# Autodesk Inventor assembly: mecanum prototype
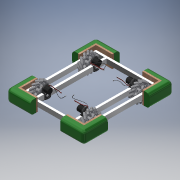
[picture p0: Inventor's stored thumbnail of the model, 180x180]
Saved by Autodesk Inventor 2018 (Build 220112000, 112)
## iProperties
Created: 2019-04-24
Part Number: mecanum prototype
Document SubType Name: Assembly
Designer: corbin
Sending System: Autodesk Inventor 2019
Preprocessor: ST-DEVELOPER v17
Title: C:\Users\corbin\Downloads\mecanum prototype.stp
Author: corbin
## Documents named in this file (10)
- C:\Users\corbin\Downloads\mecanum prototype\mecanum prototype.iam
- C:\Users\corbin\Downloads\mecanum prototype\parts\Frame Pieces\sides with bearings.iam
- C:\Users\corbin\Downloads\mecanum prototype\parts\Frame Pieces\front and back.ipt
- C:\Users\corbin\Downloads\mecanum prototype\parts\Gearbox\Single_Reduction_Clamping_Gearbox_217-4156.iam
- C:\Users\corbin\Downloads\mecanum prototype\parts\Churro.ipt
- C:\Users\corbin\Downloads\mecanum prototype\parts\REV-21-1650.ipt
- C:\Users\corbin\Downloads\mecanum prototype\parts\Wheels\8 Inch Mecanum Wheels\8_Mecanum_Wheel_Right_217-2587.iam
- C:\Users\corbin\Downloads\mecanum prototype\parts\Wheels\8 Inch Mecanum Wheels\8_Mecanum_Wheel_Left_217-2801.iam
- C:\Users\corbin\Downloads\mecanum prototype\parts\Frame Pieces\outsides.ipt
- C:\Users\corbin\Downloads\mecanum prototype\parts\bumpers.ipt
## Components (26 placed, 9 different names)
1. sides with bearings:1 [sub-assembly] — Flush:6, Mate:13, Mate:21, Mate:23, Mate:24, Mate:26, Mate:30, Flush:16, Mate:31, Flush:17
2. sides with bearings:4 [sub-assembly] — Mate:7, Flush:8, Mate:8, Flush:13, Mate:14, Mate:15, Mate:16, Mate:19, Mate:20, Mate:25, Mate:27, Mate:28, Flush:14, Mate:29, Flush:15
3. front and back:1 — Mate:6, Mate:7, Flush:8, Flush:9, Mate:11, Flush:12
4. front and back:2 — Mate:1, Flush:1, Flush:2, Mate:2, Flush:3, Flush:4, Mate:3, Flush:5, Flush:6, Flush:10, Mate:8, Mate:10, Flush:11, Flush:13
5. Single_Reduction_Clamping_Gearbox_217-4156:1 [sub-assembly] — Mate:21, Mate:23, Mate:24
6. Single_Reduction_Clamping_Gearbox_217-4156:2 [sub-assembly] — Mate:26
7. Single_Reduction_Clamping_Gearbox_217-4156:4 [sub-assembly] — Mate:19, Mate:20, Mate:27
8. Churro:1 — Mate:28, Flush:14
9. Churro:2 — Mate:29, Flush:15
10. Churro:3 — Mate:30, Flush:16
11. Churro:4 — Mate:31, Flush:17
12. REV-21-1650:1
13. REV-21-1650:2
14. REV-21-1650:3
15. REV-21-1650:4
16. Single_Reduction_Clamping_Gearbox_217-4156:5 [sub-assembly] — Mate:15, Mate:16, Mate:25
17. 8_Mecanum_Wheel_Right_217-2587:1 [sub-assembly]
18. 8_Mecanum_Wheel_Right_217-2587:2 [sub-assembly]
19. 8_Mecanum_Wheel_Left_217-2801:1 [sub-assembly]
20. 8_Mecanum_Wheel_Left_217-2801:2 [sub-assembly]
21. outsides:1 — Mate:1, Flush:1, Flush:2, Flush:10, Mate:9, Mate:12, Mate:14
22. outsides:2 — Mate:2, Flush:3, Flush:4, Mate:4, Mate:5, Flush:7, Flush:9, Mate:13
23. bumpers:1 — Mate:3, Mate:4, Flush:5
24. bumpers:2 — Mate:5, Mate:6, Flush:7
25. bumpers:3 — Mate:11, Mate:12, Flush:12
26. bumpers:4 — Mate:9, Mate:10, Flush:11
## Relationships (45: Mate 28, Flush 17)
- Mate:1: front and back:2 ↔ outsides:1
- Flush:1: front and back:2 ↔ outsides:1
- Flush:2: front and back:2 ↔ outsides:1
- Mate:2: front and back:2 ↔ outsides:2
- Flush:3: front and back:2 ↔ outsides:2
- Flush:4: front and back:2 ↔ outsides:2
- Mate:3: front and back:2 ↔ bumpers:1
- Mate:4: outsides:2 ↔ bumpers:1
- Flush:5 (-44.45 mm): front and back:2 ↔ bumpers:1
- Mate:5: outsides:2 ↔ bumpers:2
- Flush:6: sides with bearings:1 ↔ front and back:2
- Mate:6: front and back:1 ↔ bumpers:2
- Flush:7 (44.45 mm): outsides:2 ↔ bumpers:2
- Mate:7: sides with bearings:4 ↔ front and back:1
- Flush:8: sides with bearings:4 ↔ front and back:1
- Flush:9: front and back:1 ↔ outsides:2
- Flush:10: front and back:2 ↔ outsides:1
- Mate:8: sides with bearings:4 ↔ front and back:2
- Mate:9: outsides:1 ↔ bumpers:4
- Mate:10: front and back:2 ↔ bumpers:4
- Flush:11 (-44.45 mm): front and back:2 ↔ bumpers:4
- Mate:11: front and back:1 ↔ bumpers:3
- Mate:12: outsides:1 ↔ bumpers:3
- Flush:12 (44.45 mm): front and back:1 ↔ bumpers:3
- Flush:13: sides with bearings:4 ↔ front and back:2
- Mate:13 (91.44 mm): sides with bearings:1 ↔ outsides:2
- Mate:14 (91.44 mm): sides with bearings:4 ↔ outsides:1
- Mate:15: sides with bearings:4 ↔ Single_Reduction_Clamping_Gearbox_217-4156:5
- Mate:16: sides with bearings:4 ↔ Single_Reduction_Clamping_Gearbox_217-4156:5
- Mate:19: sides with bearings:4 ↔ Single_Reduction_Clamping_Gearbox_217-4156:4
- Mate:20: sides with bearings:4 ↔ Single_Reduction_Clamping_Gearbox_217-4156:4
- Mate:21: sides with bearings:1 ↔ Single_Reduction_Clamping_Gearbox_217-4156:1
- Mate:23: sides with bearings:1 ↔ Single_Reduction_Clamping_Gearbox_217-4156:1
- Mate:24: sides with bearings:1 ↔ Single_Reduction_Clamping_Gearbox_217-4156:1
- Mate:25: sides with bearings:4 ↔ Single_Reduction_Clamping_Gearbox_217-4156:5
- Mate:26: sides with bearings:1 ↔ Single_Reduction_Clamping_Gearbox_217-4156:2
- Mate:27: sides with bearings:4 ↔ Single_Reduction_Clamping_Gearbox_217-4156:4
- Mate:28: sides with bearings:4 ↔ Churro:1
- Flush:14 (-12.7 mm): sides with bearings:4 ↔ Churro:1
- Mate:29: sides with bearings:4 ↔ Churro:2
- Flush:15 (-12.7 mm): sides with bearings:4 ↔ Churro:2
- Mate:30: sides with bearings:1 ↔ Churro:3
- Flush:16 (-12.7 mm): sides with bearings:1 ↔ Churro:3
- Mate:31: sides with bearings:1 ↔ Churro:4
- Flush:17 (-12.7 mm): sides with bearings:1 ↔ Churro:4
